# Autodesk Inventor assembly: Avionics
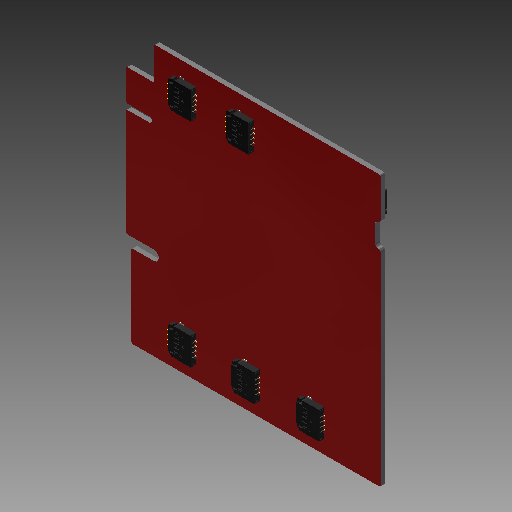
[picture p0: Inventor's stored thumbnail of the model, 512x512]
Saved by Autodesk Inventor 2018 (Build 220112000, 112)
## iProperties
Created: 2020-10-20
Part Number: Avionics
Document SubType Name: Assembly
Designer: Bradley
Author: Bradley
## Documents named in this file (4)
- C:\Users\Bradley\Documents\GitHub\CougSat1-Hardware\CougSat1-AvionicBoard\CADModel\Native\Avionics.iam
- C:\Users\Bradley\Documents\GitHub\CougSat1-Hardware\CougSat1-AvionicBoard\CADModel\Native\Avionics_PCB.ipt
- C:\Users\Bradley\Documents\GitHub\Resources\SupplierDocuments\04 - Connectors SMT\04-0001\04-0001.iam
- C:\Users\Bradley\Documents\GitHub\Resources\SupplierDocuments\04 - Connectors SMT\04-0008\04-0008.iam
## Components (8 placed, 3 different names)
1. Avionics_PCB:1 — Mate:1, Mate:2, Mate:3, Mate:4, Mate:5, Mate:6, Mate:7
2. 04-0001:1 [sub-assembly] — Mate:1, Flush:1, Mate:8
3. 04-0001:2 [sub-assembly] — Mate:2, Flush:2, Mate:9
4. 04-0001:3 [sub-assembly] — Mate:3, Flush:3, Mate:10
5. 04-0001:4 [sub-assembly] — Mate:4, Flush:4, Mate:11
6. 04-0001:5 [sub-assembly] — Mate:5, Flush:5, Mate:12
7. 04-0001:6 [sub-assembly] — Mate:6, Flush:6, Mate:13
8. 04-0008:1 [sub-assembly] — Mate:7, Flush:7, Mate:14
## Relationships (21: Mate 14, Flush 7)
- Mate:1: Avionics_PCB:1 ↔ 04-0001:1
- Mate:2: Avionics_PCB:1 ↔ 04-0001:2
- Mate:3: Avionics_PCB:1 ↔ 04-0001:3
- Mate:4: Avionics_PCB:1 ↔ 04-0001:4
- Mate:5: Avionics_PCB:1 ↔ 04-0001:5
- Mate:6: Avionics_PCB:1 ↔ 04-0001:6
- Mate:7: Avionics_PCB:1 ↔ 04-0008:1
- Flush:1 (38 mm): 04-0001:1
- Flush:2 (38 mm): 04-0001:2
- Flush:3 (38 mm): 04-0001:3
- Flush:4 (-37.5 mm): 04-0001:4
- Flush:5 (-37.6 mm): 04-0001:5
- Mate:8 (25 mm): 04-0001:1
- Mate:9 (47.5 mm): 04-0001:2
- Mate:10 (70.5 mm): 04-0001:3
- Mate:11 (25 mm): 04-0001:4
- Mate:12 (45.5 mm): 04-0001:5
- Flush:6 (-84.2 mm): 04-0001:6
- Mate:13 (41 mm): 04-0001:6
- Flush:7 (12.1 mm): 04-0008:1
- Mate:14 (76.8 mm): 04-0008:1
